# Autodesk Inventor assembly: Transmisión de correas síncronas
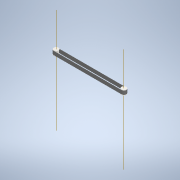
[picture p0: Inventor's stored thumbnail of the model, 180x180]
Saved by Autodesk Inventor 2021 (Build 250183000, 183)
## iProperties
ClientObjectVersion: 1
Created: 2022-10-24
Part Number: Transmisión de correas síncronas
Document SubType Name: Assembly
Designer: ivanm
Author: ivanm
## Documents named in this file (4)
- C:\Users\ivanm\OneDrive\Servomecanismos\Proyectos\Proyecto academico\Servomecanismo2R\INVENTOR\Ensamblaje\Design Accelerator\Transmisión de correas síncronas2.iam
- C:\Users\ivanm\OneDrive\Servomecanismos\Proyectos\Proyecto academico\Servomecanismo2R\INVENTOR\Ensamblaje\Design Accelerator\Correa síncrona2.ipt
- C:\Users\ivanm\OneDrive\Servomecanismos\Proyectos\Proyecto academico\Servomecanismo2R\INVENTOR\Ensamblaje\Design Accelerator\Polea síncrona11.ipt
- C:\Users\ivanm\OneDrive\Servomecanismos\Proyectos\Proyecto academico\Servomecanismo2R\INVENTOR\Ensamblaje\Design Accelerator\Polea síncrona21.ipt
## Components (3 placed, 3 different names)
1. Correa síncrona:1 — Nivelación:1, Coincidencia:1, Coincidencia:2, Nivelación:2, Coincidencia:3, Coincidencia:4
2. Polea síncrona1:1 — Nivelación:1, Coincidencia:1, Coincidencia:2, Rotación:1
3. Polea síncrona2:1 — Nivelación:2, Coincidencia:3, Rotación:1, Coincidencia:4
## Relationships (7: Mate 4, Flush 2, RelateRotation 1)
- Nivelación:1 [Flush]: Correa síncrona:1 ↔ Polea síncrona1:1
- Coincidencia:1 [Mate]: Correa síncrona:1 ↔ Polea síncrona1:1
- Coincidencia:2 [Mate]: Correa síncrona:1 ↔ Polea síncrona1:1
- Nivelación:2 [Flush]: Correa síncrona:1 ↔ Polea síncrona2:1
- Coincidencia:3 [Mate]: Correa síncrona:1 ↔ Polea síncrona2:1
- Rotación:1 [RelateRotation] (1 ul): Polea síncrona1:1 ↔ Polea síncrona2:1
- Coincidencia:4 [Mate]: Correa síncrona:1 ↔ Polea síncrona2:1
